# Autodesk Inventor assembly: s-assy-ring_gear-long
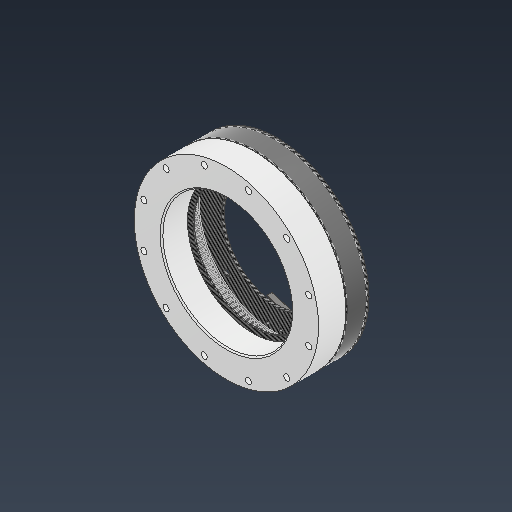
[picture p0: Inventor's stored thumbnail of the model, 512x512]
Saved by Autodesk Inventor 2021 (Build 250183000, 183)
## iProperties
Created: 2021-07-12
Part Number: s-assy-ring_gear-long
Document SubType Name: Assembly
Designer: yuta0
Mass: 191.026 g
Surface Area: 857.074 cm^2
Volume: 171.825 cm^3
Density: 1.11175 g/cm^3
Author: yuta0
## Documents named in this file (6)
- C:\Users\yuta0\Desktop\catchrobo_robot\s-assy-ring_gear-long.iam
- C:\Users\yuta0\Desktop\catchrobo_robot\base33.ipt
- C:\Users\yuta0\Desktop\catchrobo_robot\carbon_plate13.ipt
- C:\Users\yuta0\Desktop\catchrobo_robot\base27.ipt
- C:\Users\yuta0\Desktop\catchrobo_robot\carbon_plate9.ipt
- C:\Users\yuta0\Desktop\catchrobo_robot\SS-5GL.iam
## Components (5 placed, 5 different names)
1. unit-ring_gear:1 — フラッシュ:2, メイト:5, メイト:6, メイト:11, メイト:25, メイト:29
2. unit-plate3:1 — メイト:4, メイト:5, メイト:6, メイト:12, メイト:22
3. unit-base3:1 — メイト:11, メイト:12, メイト:24
4. unit-j2-plate1:1 — メイト:21, メイト:25, メイト:26, メイト:27, メイト:28, メイト:29
5. SS-5GL:1 [sub-assembly] — メイト:26, メイト:27, メイト:28
## Relationships (14: Mate 13, Flush 1)
- フラッシュ:2 [Flush]: unit-ring_gear:1
- メイト:4 [Mate]: unit-plate3:1
- メイト:5 [Mate]: unit-ring_gear:1 ↔ unit-plate3:1
- メイト:6 [Mate]: unit-ring_gear:1 ↔ unit-plate3:1
- メイト:11 [Mate]: unit-ring_gear:1 ↔ unit-base3:1
- メイト:12 [Mate]: unit-plate3:1 ↔ unit-base3:1
- メイト:21 [Mate]: unit-j2-plate1:1
- メイト:22 [Mate]: unit-plate3:1
- メイト:24 [Mate]: unit-base3:1
- メイト:25 [Mate]: unit-ring_gear:1 ↔ unit-j2-plate1:1
- メイト:26 [Mate]: unit-j2-plate1:1 ↔ SS-5GL:1
- メイト:27 [Mate]: unit-j2-plate1:1 ↔ SS-5GL:1
- メイト:28 [Mate]: unit-j2-plate1:1 ↔ SS-5GL:1
- メイト:29 [Mate]: unit-ring_gear:1 ↔ unit-j2-plate1:1
